# Autodesk Inventor assembly: Logitech_C920
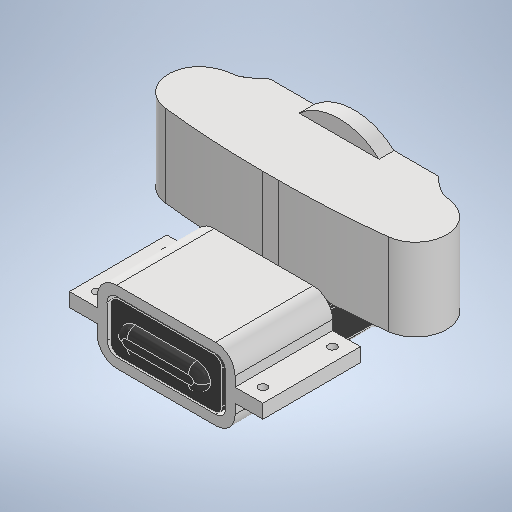
[picture p0: Inventor's stored thumbnail of the model, 512x512]
Saved by Autodesk Inventor 2025.1 (Build 291241000, 241)
## iProperties
Created: 2025-06-15
Part Number: Logitech_C920
Document SubType Name: Assembly
Designer: User
Author: User
## Documents named in this file (6)
- D:\One Drive\OneDrive - Politeknik Sultan Salahuddin Abdul Aziz Shah\Documents\Inventor\RobosotPSA\Logitech_C920.iam
- D:\One Drive\OneDrive - Politeknik Sultan Salahuddin Abdul Aziz Shah\Documents\Inventor\RobosotPSA\Logitech_C920\Logitech_C920\Logitech_C920.ipt
- D:\One Drive\OneDrive - Politeknik Sultan Salahuddin Abdul Aziz Shah\Documents\Inventor\RobosotPSA\Logitech_C920Arm\Logitech_C920Arm\Logitech_C920Arm.ipt
- D:\One Drive\OneDrive - Politeknik Sultan Salahuddin Abdul Aziz Shah\Documents\Inventor\RobosotPSA\Logitech_C920Glass\Logitech_C920Glass\Logitech_C920Glass.ipt
- D:\One Drive\OneDrive - Politeknik Sultan Salahuddin Abdul Aziz Shah\Documents\Inventor\RobosotPSA\camHolder.ipt
- D:\One Drive\OneDrive - Politeknik Sultan Salahuddin Abdul Aziz Shah\Documents\Inventor\RobosotPSA\LensHolder.ipt
## Components (5 placed, 5 different names)
1. Logitech_C920:1 — Mate:1, Flush:1, Mate:2, Mate:3, Flush:3
2. Logitech_C920Arm:1 — Mate:2, Mate:3, Flush:2
3. Logitech_C920Glass:1 — Mate:1, Flush:1
4. camHolder:1 — Flush:2
5. LensHolder:1 — Flush:3
## Relationships (6: Mate 3, Flush 3)
- Mate:1: Logitech_C920:1 ↔ Logitech_C920Glass:1
- Flush:1: Logitech_C920:1 ↔ Logitech_C920Glass:1
- Mate:2: Logitech_C920:1 ↔ Logitech_C920Arm:1
- Mate:3: Logitech_C920:1 ↔ Logitech_C920Arm:1
- Flush:2: Logitech_C920Arm:1 ↔ camHolder:1
- Flush:3: Logitech_C920:1 ↔ LensHolder:1
